# Autodesk Inventor assembly: SAFRS-A-0008
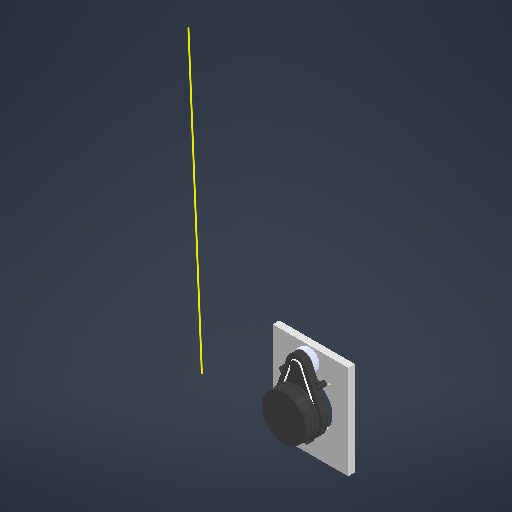
[picture p0: Inventor's stored thumbnail of the model, 512x512]
Saved by Autodesk Inventor 2026.2 (Build 302298000, 298)
## iProperties
Created: 2025-12-01
Part Number: SAFRS-A-0008
Document SubType Name: Assembly
Designer: jaewook
Author: jaewook
Title: Lidar Base Assembly
## Documents named in this file (3)
- C:\Users\jk000\OneDrive\Desktop\git\SAFRS\mechanical\inventor\02__subassemblies\lidar_base.iam
- C:\Users\jk000\OneDrive\Desktop\git\SAFRS\mechanical\inventor\01_parts\lidar_mount.ipt
- C:\Users\jk000\OneDrive\Desktop\git\SAFRS\mechanical\inventor\01_parts\ydlidar_x4_pro.ipt
## Components (2 placed, 2 different names)
1. Lidar_base:1 — 메이트:1
2. ydlidar_x4_pro:1 — 메이트:1
## Relationships (1: Mate 1)
- 메이트:1 [Mate]: Lidar_base:1 ↔ ydlidar_x4_pro:1
